# Autodesk Inventor assembly: Tall Conveyor-Belt Link
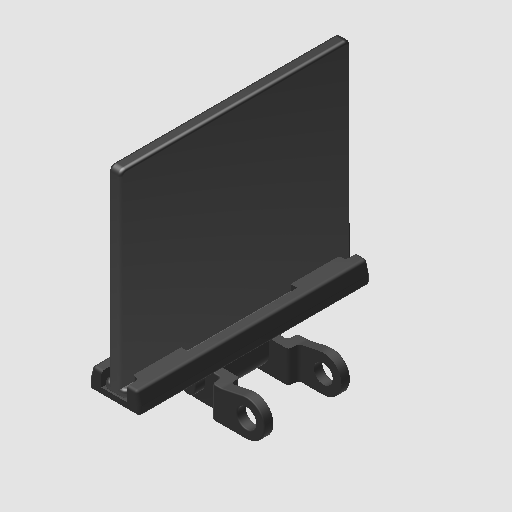
[picture p0: Inventor's stored thumbnail of the model, 512x512]
Saved by Autodesk Inventor 2019.3 (Build 233278000, 278)
## iProperties
Category: Motion
Company: Super Sonic Sparks, Team 24
Vendor: VEX Robotics, Inc.
Document SubType Name: Assembly
Designer: Jordan Kiesel
Catalog Web Link: vexrobotics.com/276-2214.html
Description: For use in constructing conveyor belt type mechanisms.
Part Number: Tall Conveyor-Belt Link
Mass: 4.00785 g
Surface Area: 45.192 cm^2
Volume: 3.69222 cm^3
Density: 1.08549 g/cm^3
Created: 2018-08-26
Author: Jordan Kiesel
Title: Medium Conveyor-Belt Link
Comments: For use in constructing conveyor belt type mechanisms. ▷ Compatible with Tank Tread Kit, High Strength Chain & Sprockets.
## Documents named in this file (3)
- D:\vex cad\零件库\履带链条\Tall Conveyor-Belt Link.iam
- D:\vex cad\零件库\履带链条\Reference Parts\Conveyor-Belt Links\Conveyor-Belt Base Link.ipt
- D:\vex cad\零件库\履带链条\Reference Parts\Conveyor-Belt Links\Tall Conveyor-Belt Insert.ipt
## Components (2 placed, 2 different names)
1. Conveyor-Belt Base Link:1 — Mate:1, Mate:2, Flush:1
2. Tall Conveyor-Belt Insert:1 — Mate:1, Mate:2, Flush:1
## Relationships (3: Mate 2, Flush 1)
- Mate:1: Conveyor-Belt Base Link:1 ↔ Tall Conveyor-Belt Insert:1
- Mate:2: Conveyor-Belt Base Link:1 ↔ Tall Conveyor-Belt Insert:1
- Flush:1: Conveyor-Belt Base Link:1 ↔ Tall Conveyor-Belt Insert:1
